# Autodesk Inventor assembly: Assembly5
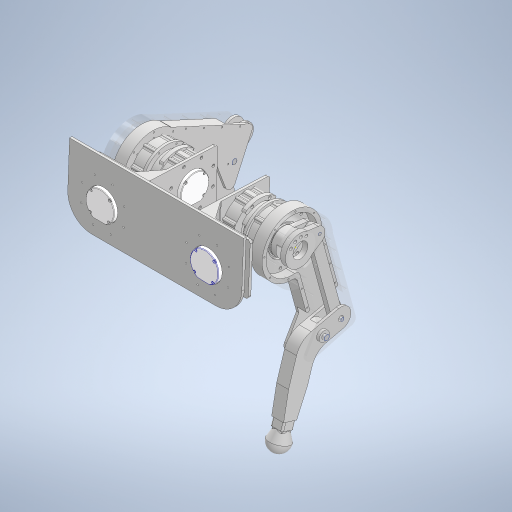
[picture p0: Inventor's stored thumbnail of the model, 512x512]
Saved by Autodesk Inventor 2024.3 (Build 283343000, 343)
## iProperties
Created: 2025-01-16
Part Number: Assembly5
Document SubType Name: Assembly
Designer: 佐藤智貴
Author: 佐藤智貴
## Documents named in this file (32)
- C:\Users\佐藤智貴\OneDrive - Chiba Institute of Technology\ドキュメント\Inventor\Biped_robot\Assembly5.iam
- C:\Users\佐藤智貴\OneDrive - Chiba Institute of Technology\ドキュメント\Inventor\Biped_robot\legparts_06(six).ipt
- C:\Users\佐藤智貴\OneDrive - Chiba Institute of Technology\ドキュメント\Inventor\Biped_robot\legparts_08(six).ipt
- C:\Users\佐藤智貴\OneDrive - Chiba Institute of Technology\ドキュメント\Inventor\Biped_robot\sole05.ipt
- C:\Users\佐藤智貴\OneDrive - Chiba Institute of Technology\ドキュメント\Inventor\Biped_robot\8108-8.iam
- C:\Users\佐藤智貴\OneDrive - Chiba Institute of Technology\ドキュメント\Inventor\Biped_robot\legparts_03(six).ipt
- C:\Users\佐藤智貴\OneDrive - Chiba Institute of Technology\ドキュメント\Inventor\Biped_robot\10mm_bearing.ipt
- C:\Users\佐藤智貴\OneDrive - Chiba Institute of Technology\ドキュメント\Inventor\Biped_robot\legparts_01.ipt
- C:\Users\佐藤智貴\OneDrive - Chiba Institute of Technology\ドキュメント\Inventor\Biped_robot\legparts_10.ipt
- C:\Users\佐藤智貴\OneDrive - Chiba Institute of Technology\ドキュメント\Inventor\Biped_robot\legparts_07(four).ipt
- C:\Users\佐藤智貴\OneDrive - Chiba Institute of Technology\ドキュメント\Inventor\Biped_robot\legparts_08(six)_MIR.ipt
- C:\Users\佐藤智貴\OneDrive - Chiba Institute of Technology\ドキュメント\Inventor\Biped_robot\3.5mm_spacer.ipt
- C:\Users\佐藤智貴\OneDrive - Chiba Institute of Technology\ドキュメント\Inventor\Biped_robot\shaft10_30mm.ipt
- C:\Users\佐藤智貴\OneDrive - Chiba Institute of Technology\ドキュメント\Inventor\Biped_robot\shaft10_45mm.ipt
- C:\Users\佐藤智貴\OneDrive - Chiba Institute of Technology\ドキュメント\Inventor\Biped_robot\legparts_09(six).ipt
- C:\Users\佐藤智貴\OneDrive - Chiba Institute of Technology\ドキュメント\Inventor\Biped_robot\legparts_02(six).ipt
- C:\Users\佐藤智貴\OneDrive - Chiba Institute of Technology\ドキュメント\Inventor\Biped_robot\legparts_04(six).ipt
- C:\Users\佐藤智貴\OneDrive - Chiba Institute of Technology\ドキュメント\Inventor\Biped_robot\legparts_06(six)_MIR1.ipt
- C:\Users\佐藤智貴\OneDrive - Chiba Institute of Technology\ドキュメント\Inventor\Biped_robot\legparts_08(six)_MIR2.ipt
- C:\Users\佐藤智貴\OneDrive - Chiba Institute of Technology\ドキュメント\Inventor\Biped_robot\sole05_MIR1.ipt
- C:\Users\佐藤智貴\OneDrive - Chiba Institute of Technology\ドキュメント\Inventor\Biped_robot\8108-8_MIR4.iam
- C:\Users\佐藤智貴\OneDrive - Chiba Institute of Technology\ドキュメント\Inventor\Biped_robot\legparts_03(six)_MIR1.ipt
- C:\Users\佐藤智貴\OneDrive - Chiba Institute of Technology\ドキュメント\Inventor\Biped_robot\10mm_bearing_MIR2.ipt
- C:\Users\佐藤智貴\OneDrive - Chiba Institute of Technology\ドキュメント\Inventor\Biped_robot\legparts_01_MIR3.ipt
- C:\Users\佐藤智貴\OneDrive - Chiba Institute of Technology\ドキュメント\Inventor\Biped_robot\legparts_10_MIR1.ipt
- C:\Users\佐藤智貴\OneDrive - Chiba Institute of Technology\ドキュメント\Inventor\Biped_robot\legparts_07(four)_MIR2.ipt
- C:\Users\佐藤智貴\OneDrive - Chiba Institute of Technology\ドキュメント\Inventor\Biped_robot\legparts_08(six)_MIR_MIR1.ipt
- C:\Users\佐藤智貴\OneDrive - Chiba Institute of Technology\ドキュメント\Inventor\Biped_robot\3.5mm_spacer_MIR1.ipt
- C:\Users\佐藤智貴\OneDrive - Chiba Institute of Technology\ドキュメント\Inventor\Biped_robot\shaft10_30mm_MIR2.ipt
- C:\Users\佐藤智貴\OneDrive - Chiba Institute of Technology\ドキュメント\Inventor\Biped_robot\shaft10_45mm_MIR1.ipt
- C:\Users\佐藤智貴\OneDrive - Chiba Institute of Technology\ドキュメント\Inventor\Biped_robot\legparts_02(six)_MIR.ipt
- C:\Users\佐藤智貴\OneDrive - Chiba Institute of Technology\ドキュメント\Inventor\Biped_robot\legparts_04(six)_MIR.ipt
## Components (47 placed, 31 different names)
1. legparts_06(six):1 — 挿入:1, メイト:1, 挿入:11, 挿入:12, 挿入:25, 挿入:31, 挿入:32, 挿入:34
2. legparts_08(six):2 — 挿入:2, 挿入:25, 挿入:69, 挿入:70
3. sole05:1 — 挿入:1, メイト:1
4. 8108-8:1 [sub-assembly] — 挿入:2, 挿入:13, 挿入:14, 挿入:75, 挿入:78
5. 8108-8:2 [sub-assembly] — 挿入:22, 挿入:67
6. 8108-8:3 [sub-assembly] — 挿入:15, 挿入:20, 挿入:21, 挿入:27, 挿入:28, 挿入:29, 挿入:30
7. legparts_03(six):1 — 挿入:6, 挿入:7, 挿入:9, 挿入:10
8. 10mm_bearing:1 — 挿入:6
9. 10mm_bearing:2 — 挿入:7, 挿入:77
10. 10mm_bearing:3 — 挿入:10, 挿入:11
11. 10mm_bearing:4 — 挿入:9, 挿入:12
12. legparts_01:1 — 挿入:13, 挿入:14, 挿入:15
13. legparts_10:1 — 挿入:29, 挿入:30
14. legparts_10:2 — 挿入:27, 挿入:28
15. legparts_07(four):1 — 挿入:20, 挿入:21, 挿入:22
16. legparts_08(six)_MIR:1 — 挿入:35, 挿入:69, 挿入:70
17. 3.5mm_spacer:1 — 挿入:31
18. 3.5mm_spacer:2 — 挿入:32
19. shaft10_30mm:1 — 挿入:76
20. shaft10_30mm:2 — 挿入:34
21. shaft10_45mm:1 — 挿入:35
22. legparts_09(six):1 — 挿入:67, 挿入:110, 挿入:111
23. legparts_02(six):1 — 挿入:73, 挿入:74, 挿入:75, 挿入:78
24. legparts_04(six):1 — 挿入:73, 挿入:74, 挿入:76, 挿入:77
25. legparts_06(six)_MIR1:1 — 挿入:79, メイト:2, 挿入:80, 挿入:84, 挿入:86, 挿入:100, 挿入:101, 挿入:102
26. legparts_08(six)_MIR2:1 — 挿入:79, 挿入:81, 挿入:98, 挿入:99
27. sole05_MIR1:1 — メイト:2, 挿入:80
28. 8108-8_MIR4:1 [sub-assembly] — 挿入:81, 挿入:89, 挿入:90, 挿入:104, 挿入:105
29. 8108-8_MIR4:2 [sub-assembly] — 挿入:95, 挿入:110, 挿入:111
30. 8108-8_MIR4:3 [sub-assembly] — 挿入:88, 挿入:91, 挿入:92, 挿入:93, 挿入:94, 挿入:96, 挿入:97
31. legparts_03(six)_MIR1:1 — 挿入:82, 挿入:83, 挿入:85, 挿入:87
32. 10mm_bearing_MIR2:1 — 挿入:82
33. 10mm_bearing_MIR2:2 — 挿入:83, 挿入:106
34. 10mm_bearing_MIR2:3 — 挿入:84, 挿入:85
35. 10mm_bearing_MIR2:4 — 挿入:86, 挿入:87
36. legparts_01_MIR3:1 — 挿入:88, 挿入:89, 挿入:90
37. legparts_10_MIR1:1 — 挿入:91, 挿入:92
38. legparts_10_MIR1:2 — 挿入:93, 挿入:94
39. legparts_07(four)_MIR2:1 — 挿入:95, 挿入:96, 挿入:97
40. legparts_08(six)_MIR_MIR1:1 — 挿入:98, 挿入:99, 挿入:103
41. 3.5mm_spacer_MIR1:1 — 挿入:100
42. 3.5mm_spacer_MIR1:2 — 挿入:101
43. shaft10_30mm_MIR2:1 — 挿入:107
44. shaft10_30mm_MIR2:2 — 挿入:102
45. shaft10_45mm_MIR1:1 — 挿入:103
46. legparts_02(six)_MIR:1 — 挿入:104, 挿入:105, 挿入:108, 挿入:109
47. legparts_04(six)_MIR:1 — 挿入:106, 挿入:107, 挿入:108, 挿入:109
## Relationships (67: Insert 65, Mate 2)
- 挿入:1 [Insert]: legparts_06(six):1 ↔ sole05:1
- メイト:1 [Mate]: legparts_06(six):1 ↔ sole05:1
- 挿入:2 [Insert]: legparts_08(six):2 ↔ 8108-8:1
- 挿入:6 [Insert]: legparts_03(six):1 ↔ 10mm_bearing:1
- 挿入:7 [Insert]: legparts_03(six):1 ↔ 10mm_bearing:2
- 挿入:9 [Insert]: legparts_03(six):1 ↔ 10mm_bearing:4
- 挿入:10 [Insert]: legparts_03(six):1 ↔ 10mm_bearing:3
- 挿入:11 [Insert]: legparts_06(six):1 ↔ 10mm_bearing:3
- 挿入:12 [Insert]: legparts_06(six):1 ↔ 10mm_bearing:4
- 挿入:13 [Insert]: 8108-8:1 ↔ legparts_01:1
- 挿入:14 [Insert]: 8108-8:1 ↔ legparts_01:1
- 挿入:15 [Insert]: 8108-8:3 ↔ legparts_01:1
- 挿入:20 [Insert]: 8108-8:3 ↔ legparts_07(four):1
- 挿入:21 [Insert]: 8108-8:3 ↔ legparts_07(four):1
- 挿入:22 [Insert]: 8108-8:2 ↔ legparts_07(four):1
- 挿入:25 [Insert] (5.5 mm): legparts_06(six):1 ↔ legparts_08(six):2
- 挿入:27 [Insert]: 8108-8:3 ↔ legparts_10:2
- 挿入:28 [Insert]: 8108-8:3 ↔ legparts_10:2
- 挿入:29 [Insert]: 8108-8:3 ↔ legparts_10:1
- 挿入:30 [Insert]: 8108-8:3 ↔ legparts_10:1
- 挿入:31 [Insert]: legparts_06(six):1 ↔ 3.5mm_spacer:1
- 挿入:32 [Insert]: legparts_06(six):1 ↔ 3.5mm_spacer:2
- 挿入:34 [Insert] (-3 mm): legparts_06(six):1 ↔ shaft10_30mm:2
- 挿入:35 [Insert]: legparts_08(six)_MIR:1 ↔ shaft10_45mm:1
- 挿入:67 [Insert]: 8108-8:2 ↔ legparts_09(six):1
- 挿入:69 [Insert]: legparts_08(six):2 ↔ legparts_08(six)_MIR:1
- 挿入:70 [Insert]: legparts_08(six):2 ↔ legparts_08(six)_MIR:1
- 挿入:73 [Insert]: legparts_02(six):1 ↔ legparts_04(six):1
- 挿入:74 [Insert]: legparts_02(six):1 ↔ legparts_04(six):1
- 挿入:75 [Insert]: 8108-8:1 ↔ legparts_02(six):1
- 挿入:76 [Insert]: shaft10_30mm:1 ↔ legparts_04(six):1
- 挿入:77 [Insert]: 10mm_bearing:2 ↔ legparts_04(six):1
- 挿入:78 [Insert]: 8108-8:1 ↔ legparts_02(six):1
- 挿入:79 [Insert] (5.5 mm): legparts_06(six)_MIR1:1 ↔ legparts_08(six)_MIR2:1
- メイト:2 [Mate]: legparts_06(six)_MIR1:1 ↔ sole05_MIR1:1
- 挿入:80 [Insert]: legparts_06(six)_MIR1:1 ↔ sole05_MIR1:1
- 挿入:81 [Insert]: legparts_08(six)_MIR2:1 ↔ 8108-8_MIR4:1
- 挿入:82 [Insert]: legparts_03(six)_MIR1:1 ↔ 10mm_bearing_MIR2:1
- 挿入:83 [Insert]: legparts_03(six)_MIR1:1 ↔ 10mm_bearing_MIR2:2
- 挿入:84 [Insert]: legparts_06(six)_MIR1:1 ↔ 10mm_bearing_MIR2:3
- 挿入:85 [Insert]: legparts_03(six)_MIR1:1 ↔ 10mm_bearing_MIR2:3
- 挿入:86 [Insert]: legparts_06(six)_MIR1:1 ↔ 10mm_bearing_MIR2:4
- 挿入:87 [Insert]: legparts_03(six)_MIR1:1 ↔ 10mm_bearing_MIR2:4
- 挿入:88 [Insert]: 8108-8_MIR4:3 ↔ legparts_01_MIR3:1
- 挿入:89 [Insert]: 8108-8_MIR4:1 ↔ legparts_01_MIR3:1
- 挿入:90 [Insert]: 8108-8_MIR4:1 ↔ legparts_01_MIR3:1
- 挿入:91 [Insert]: 8108-8_MIR4:3 ↔ legparts_10_MIR1:1
- 挿入:92 [Insert]: 8108-8_MIR4:3 ↔ legparts_10_MIR1:1
- 挿入:93 [Insert]: 8108-8_MIR4:3 ↔ legparts_10_MIR1:2
- 挿入:94 [Insert]: 8108-8_MIR4:3 ↔ legparts_10_MIR1:2
- 挿入:95 [Insert]: 8108-8_MIR4:2 ↔ legparts_07(four)_MIR2:1
- 挿入:96 [Insert]: 8108-8_MIR4:3 ↔ legparts_07(four)_MIR2:1
- 挿入:97 [Insert]: 8108-8_MIR4:3 ↔ legparts_07(four)_MIR2:1
- 挿入:98 [Insert]: legparts_08(six)_MIR2:1 ↔ legparts_08(six)_MIR_MIR1:1
- 挿入:99 [Insert]: legparts_08(six)_MIR2:1 ↔ legparts_08(six)_MIR_MIR1:1
- 挿入:100 [Insert]: legparts_06(six)_MIR1:1 ↔ 3.5mm_spacer_MIR1:1
- 挿入:101 [Insert]: legparts_06(six)_MIR1:1 ↔ 3.5mm_spacer_MIR1:2
- 挿入:102 [Insert] (-3 mm): legparts_06(six)_MIR1:1 ↔ shaft10_30mm_MIR2:2
- 挿入:103 [Insert]: legparts_08(six)_MIR_MIR1:1 ↔ shaft10_45mm_MIR1:1
- 挿入:104 [Insert]: 8108-8_MIR4:1 ↔ legparts_02(six)_MIR:1
- 挿入:105 [Insert]: 8108-8_MIR4:1 ↔ legparts_02(six)_MIR:1
- 挿入:106 [Insert]: 10mm_bearing_MIR2:2 ↔ legparts_04(six)_MIR:1
- 挿入:107 [Insert]: shaft10_30mm_MIR2:1 ↔ legparts_04(six)_MIR:1
- 挿入:108 [Insert]: legparts_02(six)_MIR:1 ↔ legparts_04(six)_MIR:1
- 挿入:109 [Insert]: legparts_02(six)_MIR:1 ↔ legparts_04(six)_MIR:1
- 挿入:110 [Insert]: legparts_09(six):1 ↔ 8108-8_MIR4:2
- 挿入:111 [Insert]: legparts_09(six):1 ↔ 8108-8_MIR4:2
